# Autodesk Inventor assembly: Funnel
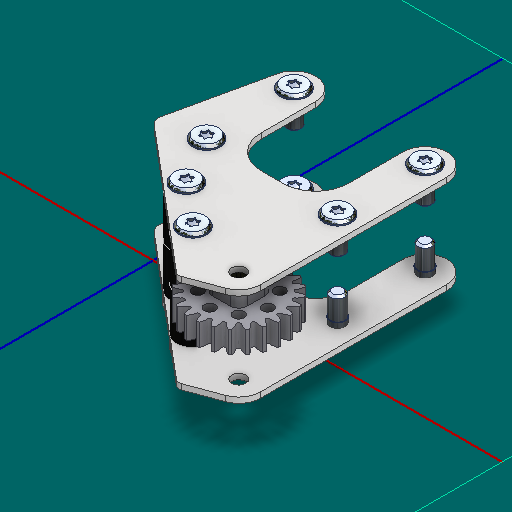
[picture p0: Inventor's stored thumbnail of the model, 512x512]
Saved by Autodesk Inventor 2025 (Build 290162000, 162)
## iProperties
Created: 2024-10-18
Part Number: Funnel
Document SubType Name: Assembly
Designer: averey
Author: averey
## Documents named in this file (11)
- C:\Users\avere\VEX\High Stakes\CAD\V2\Chassis\Drivebay Left\Funnel.iam
- C:\Users\avere\VEX\High Stakes\CAD\V2\Chassis\Drivebay Left\Custom Parts\Funnel Gusset.ipt
- C:\Users\avere\VEX\High Stakes\CAD\ROBOPROS-CAD-Inventor\Motion\Spacers\Spacer Nylon .375 OD\NSpacer .375 OD x .500.ipt
- C:\Users\avere\VEX\High Stakes\CAD\ROBOPROS-CAD-Inventor\Motion\Spacers\Spacer Nylon .375 OD.ipt
- C:\Users\avere\VEX\High Stakes\CAD\ROBOPROS-CAD-Inventor\Structure\Hardware\Screw Steel - Star\SScrew Star Smooth 1.250.ipt
- C:\Users\avere\VEX\High Stakes\CAD\ROBOPROS-CAD-Inventor\Structure\Hardware\Screw Steel - Star.ipt
- C:\Users\avere\VEX\High Stakes\CAD\ROBOPROS-CAD-Inventor\Structure\Hardware\Nut Nylon\Nut Nylon - White.ipt
- C:\Users\avere\VEX\High Stakes\CAD\ROBOPROS-CAD-Inventor\Structure\Hardware\Nut Nylon.ipt
- C:\Users\avere\VEX\High Stakes\CAD\ROBOPROS-CAD-Inventor\Structure\Hardware\Screw Shoulder Robosource\SScrew Shoulder Smooth .375 x .12.ipt
- C:\Users\avere\VEX\High Stakes\CAD\ROBOPROS-CAD-Inventor\Structure\Hardware\Screw Shoulder Robosource.ipt
- C:\Users\avere\VEX\High Stakes\CAD\ROBOPROS-CAD-Inventor\Modified Parts\Half Cut HS 24T Gear, No Insert.ipt
## Components (21 placed, 6 different names)
1. Funnel Gusset:1 — Insert:4, Insert:5, Insert:6, Insert:9, Insert:13
2. Funnel Gusset:2 — Insert:2, Insert:7, Insert:8, Insert:10, Insert:11, Insert:12
3. NSpacer .375 OD x .500:1 — Insert:1
4. NSpacer .375 OD x .500:2 — Insert:1, Insert:2
5. NSpacer .375 OD x .500:3 — Insert:4
6. NSpacer .375 OD x .500:4
7. SScrew Star Smooth 1.250:1 — Insert:5
8. SScrew Star Smooth 1.250:2 — Insert:6
9. Nut Nylon - White:1 — Insert:8
10. Nut Nylon - White:2 — Insert:7
11. SScrew Shoulder Smooth .375 x .12:9 — Insert:11
12. Nut Nylon - White:3 — Insert:12
13. Half Cut HS 24T Gear, No Insert:1 — Insert:13
14. SScrew Shoulder Smooth .375 x .12:1 — Insert:9
15. SScrew Shoulder Smooth .375 x .12:2
16. SScrew Shoulder Smooth .375 x .12:3
17. SScrew Shoulder Smooth .375 x .12:4
18. SScrew Shoulder Smooth .375 x .12:5 — Insert:10
19. SScrew Shoulder Smooth .375 x .12:6
20. SScrew Shoulder Smooth .375 x .12:7
21. SScrew Shoulder Smooth .375 x .12:8
## Component patterns: Top Mounting Screws (4 elements), Bottom Mounting Screw Pattern (4 elements)
## Relationships (14: Insert 13, Mate 1)
- [Mate]: Funnel Gusset:1 ↔ Funnel Gusset:2
- Insert:1: NSpacer .375 OD x .500:1 ↔ NSpacer .375 OD x .500:2
- Insert:2: Funnel Gusset:2 ↔ NSpacer .375 OD x .500:2
- [Insert]: NSpacer .375 OD x .500:3 ↔ NSpacer .375 OD x .500:4
- Insert:4: Funnel Gusset:1 ↔ NSpacer .375 OD x .500:3
- Insert:5: Funnel Gusset:1 ↔ SScrew Star Smooth 1.250:1
- Insert:6: Funnel Gusset:1 ↔ SScrew Star Smooth 1.250:2
- Insert:7: Funnel Gusset:2 ↔ Nut Nylon - White:2
- Insert:8: Funnel Gusset:2 ↔ Nut Nylon - White:1
- Insert:9: Funnel Gusset:1 ↔ SScrew Shoulder Smooth .375 x .12:1
- Insert:10: Funnel Gusset:2 ↔ SScrew Shoulder Smooth .375 x .12:5
- Insert:11 (1.5875 mm): Funnel Gusset:2 ↔ SScrew Shoulder Smooth .375 x .12:9
- Insert:12: Funnel Gusset:2 ↔ Nut Nylon - White:3
- Insert:13: Funnel Gusset:1 ↔ Half Cut HS 24T Gear, No Insert:1
## Named parameters: d3_d1 = 0 mm
